# Autodesk Inventor assembly: M178-2000
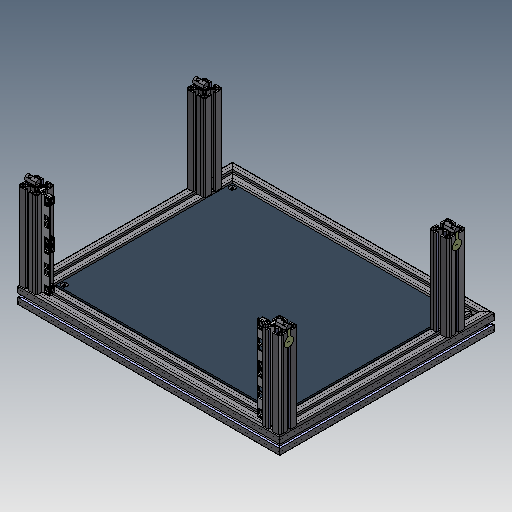
[picture p0: Inventor's stored thumbnail of the model, 512x512]
Saved by Autodesk Inventor 2018.3 (Build 223284000, 284)
## iProperties
Created: 2004-11-19
Part Number: M178-2000
Document SubType Name: Assembly
Designer: Autodesk, Inc.
Manufacturer: Standard
Standards Organization: Custom
Mass: 6108.07 g
Surface Area: 20444.6 cm^2
Volume: 3295.53 cm^3
Density: 1.85344 g/cm^3
CAGE: 1LJX3
Dept. ID: Product Design
Description #2: ---
Finish #1: ---
Finish #2: ---
Material ID: ---
Project Number: ---
Author: Autodesk, Inc.
## Documents named in this file (16)
- C:\AVAInvAPI\Workspace\Test Station\Components\M178-2000.iam
- C:\AVAInvAPI\Workspace\Test Station\Components\M178-2001.ipt
- C:\AVAInvAPI\Workspace\Test Station\Components\22-100.ipt
- C:\AVAInvAPI\Workspace\Test Station\Components\20-004.iam
- C:\AVAInvAPI\Workspace\Test Station\Components\M178-2002-01.ipt
- C:\AVAInvAPI\Workspace\Test Station\Components\M178-2002-02.ipt
- C:\AVAInvAPI\Workspace\Test Station\Components\M178-2005.ipt
- C:\AVAInvAPI\Workspace\Test Station\Components\M178-2000-Base_Phantom.iam
- C:\AVAInvAPI\Workspace\Test Station\Components\20-075.ipt
- C:\AVAInvAPI\Workspace\Test Station\Components\24-506-6F.ipt
- C:\AVAInvAPI\Workspace\Test Station\Components\24-230-6.ipt
- C:\Users\kelleyb.ADS\Desktop\Samples MIGRATED 2009 224 RTM_1\Standard Parts\Test Station Content\Extrusions\Rack Angle (19in).ipt
- C:\Users\kelleyb.ADS\Desktop\Samples MIGRATED 2009 224 RTM_1\Standard Parts\Test Station Content\Extrusions\40 Series Profiles.ipt
- C:\Users\kelleyb.ADS\Desktop\Samples MIGRATED 2009 224 RTM_1\Standard Parts\Test Station Content\Fastners\20-07X Clip Nut.ipt
- C:\Users\kelleyb.ADS\Desktop\Samples MIGRATED 2009 224 RTM_1\Standard Parts\Test Station Content\Fastners\24-5XX-YY Setscrews.ipt
- C:\Users\kelleyb.ADS\Desktop\Samples MIGRATED 2009 224 RTM_1\Standard Parts\Test Station Content\Fastners\2X-YYY-ZZ IPS Screws.ipt
## Components (37 placed, 10 different names)
1. M178-2001:1 — Flush:2, Mate:2, Flush:3, Mate:11, Insert:6, Insert:7
2. M178-2001:2 — Flush:1, Mate:2, Flush:3, Mate:3, Flush:4, Mate:4, Mate:5, Mate:10, Angle:1, Insert:4, Insert:5, Mate:19, Mate:8, Mate:9
3. M178-2000-Base_Phantom:1 [sub-assembly] — Mate:12, Flush:7, Flush:8, Flush:9, Mate:13, Mate:15, Mate:16, Mate:17, Mate:18
4. M178-2000-Base_Phantom:2 [sub-assembly] — Flush:9, Mate:13, Flush:10, Mate:14, Flush:11
5. 24-506-6F:1 — Insert:5
6. 24-506-6F:2 — Insert:4
7. 24-506-6F:3 — Insert:7
8. 24-506-6F:4 — Insert:6
9. M178-2005:1 — Flush:14, Mate:17, Mate:18, Insert:8, Insert:9, Insert:10, Insert:11
10. 24-230-6:1 — Insert:9
11. 24-230-6:2 — Insert:8
12. 24-230-6:3 — Insert:10
13. 24-230-6:4 — Insert:11
14. 20-075:2 — Flush:15, Flush:16, Mate:19
15. 20-075:1 — Mate:10, Angle:1, Flush:15, Flush:16, Mate:8, Mate:9
16. 20-075:3
17. 20-075:6
18. 20-075:4
19. 20-075:7
20. 20-075:5
21. 20-075:8
22. M178-2002-01:1 — Flush:4, Mate:4, Mate:5, Flush:5, Flush:6, Insert:1, Angle:3, Mate:12, Flush:7, Flush:8, Insert:3, Angle:4
23. 20-004:1 [sub-assembly] — Insert:1, Angle:3
24. M178-2002-02:4 — Flush:5, Flush:6, Mate:11, Insert:2, Angle:2, Flush:10
25. 20-004:2 [sub-assembly] — Insert:2, Angle:2
26. M178-2002-01:3
27. 20-004:3 [sub-assembly]
28. M178-2002-02:2
29. 20-004:4 [sub-assembly]
30. 20-004:5 [sub-assembly] — Insert:3, Angle:4
31. 20-004:6 [sub-assembly]
32. 20-004:7 [sub-assembly]
33. 20-004:8 [sub-assembly]
34. 22-100:1 — Mate:14, Mate:15, Flush:11, Flush:12, Flush:13
35. 22-100:2 — Mate:16, Flush:12, Flush:13
36. 22-100:3 — Flush:14
37. 22-100:4
## Component patterns: (4 elements, first: 20-075:2 + 20-075:1), (2 elements, first: M178-2002-01:1 + 20-004:1 + M178-2002-02:4 + 20-004:2), (4 elements, first: 20-004:5), (2 elements, first: 22-100:1 + 22-100:2)
## Relationships (48: Mate 17, Flush 16, Insert 11, Angle 4)
- Flush:1: M178-2001:2
- Flush:2: M178-2001:1
- [Mate] (-241.3 mm): M178-2001:2
- Mate:2 (-482.6 mm): M178-2001:1 ↔ M178-2001:2
- Flush:3: M178-2001:1 ↔ M178-2001:2
- Mate:3: M178-2001:2
- Flush:4: M178-2001:2 ↔ M178-2002-01:1
- Mate:4: M178-2001:2 ↔ M178-2002-01:1
- Mate:5: M178-2001:2 ↔ M178-2002-01:1
- Mate:10: M178-2001:2 ↔ 20-075:1
- Angle:1 (0 deg): M178-2001:2 ↔ 20-075:1
- Flush:5: M178-2002-01:1 ↔ M178-2002-02:4
- Flush:6: M178-2002-01:1 ↔ M178-2002-02:4
- Mate:11: M178-2001:1 ↔ M178-2002-02:4
- Insert:1: M178-2002-01:1 ↔ 20-004:1
- Insert:2: M178-2002-02:4 ↔ 20-004:2
- Angle:2 (0 deg): M178-2002-02:4 ↔ 20-004:2
- Angle:3 (0 deg): M178-2002-01:1 ↔ 20-004:1
- Mate:12: M178-2000-Base_Phantom:1 ↔ M178-2002-01:1
- Flush:7: M178-2000-Base_Phantom:1 ↔ M178-2002-01:1
- Flush:8: M178-2000-Base_Phantom:1 ↔ M178-2002-01:1
- Flush:9: M178-2000-Base_Phantom:1 ↔ M178-2000-Base_Phantom:2
- Mate:13: M178-2000-Base_Phantom:1 ↔ M178-2000-Base_Phantom:2
- Flush:10: M178-2000-Base_Phantom:2 ↔ M178-2002-02:4
- Insert:3: M178-2002-01:1 ↔ 20-004:5
- Angle:4 (0 deg): M178-2002-01:1 ↔ 20-004:5
- Insert:4: M178-2001:2 ↔ 24-506-6F:2
- Insert:5: M178-2001:2 ↔ 24-506-6F:1
- Insert:6: M178-2001:1 ↔ 24-506-6F:4
- Insert:7: M178-2001:1 ↔ 24-506-6F:3
- Mate:14: M178-2000-Base_Phantom:2 ↔ 22-100:1
- Mate:15: M178-2000-Base_Phantom:1 ↔ 22-100:1
- Flush:11 (10 mm): M178-2000-Base_Phantom:2 ↔ 22-100:1
- Mate:16: M178-2000-Base_Phantom:1 ↔ 22-100:2
- Flush:12: 22-100:1 ↔ 22-100:2
- Flush:13: 22-100:1 ↔ 22-100:2
- Flush:14: M178-2005:1 ↔ 22-100:3
- Mate:17 (1.27 mm): M178-2000-Base_Phantom:1 ↔ M178-2005:1
- Mate:18 (1.27 mm): M178-2000-Base_Phantom:1 ↔ M178-2005:1
- Insert:8: M178-2005:1 ↔ 24-230-6:2
- Insert:9: M178-2005:1 ↔ 24-230-6:1
- Insert:10: M178-2005:1 ↔ 24-230-6:3
- Insert:11: M178-2005:1 ↔ 24-230-6:4
- Flush:15: 20-075:2 ↔ 20-075:1
- Flush:16: 20-075:2 ↔ 20-075:1
- Mate:19 (4.7625 mm): M178-2001:2 ↔ 20-075:2
- Mate:8 (4.75 mm): M178-2001:2 ↔ 20-075:1
- Mate:9 (4.75 mm): M178-2001:2 ↔ 20-075:1
